# Autodesk Inventor assembly: KB33-046-002 - Привод в сборе
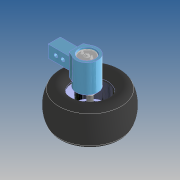
[picture p0: Inventor's stored thumbnail of the model, 180x180]
Saved by Autodesk Inventor 2020 (Build 240168000, 168)
## iProperties
Created: 2021-06-21
Part Number: KB33-046-002 - Привод в сборе
Document SubType Name: Assembly
Designer: Петров Иван
Mass: 1171.6 g
Surface Area: 1587.77 cm^2
Volume: 1165.85 cm^3
Density: 1.00493 g/cm^3
Author: Петров Иван
## Documents named in this file (6)
- E:\IVAN\Ivan_desktop\Kvantorium\Projects\RoboPatrol\design\KB33-046-002 - Привод в сборе.iam
- E:\IVAN\Ivan_desktop\Kvantorium\Projects\RoboPatrol\design\KB33-046-002-001 - Крепление.ipt
- E:\IVAN\Ivan_desktop\Kvantorium\Projects\RoboPatrol\design\standart_components\dc_gear_motor_12V_500rpm\dc_gear_motor_12V_500rpm.ipt
- E:\IVAN\Ivan_desktop\Kvantorium\Projects\RoboPatrol\design\standart_components\WheelBig\колесо большое1.iam
- E:\IVAN\Ivan_desktop\Kvantorium\Projects\RoboPatrol\design\KB33-046-002-002 - Втулка.ipt
- E:\IVAN\Ivan_desktop\Kvantorium\Projects\RoboPatrol\design\KB33-046-002-003 - Фиксирующая гайка.ipt
## Components (6 placed, 5 different names)
1. KB33-046-002-001 - Крепление:1 — Заподлицо:1, Совмещение:1, Совмещение:2
2. dc_gear_motor_12V_500rpm:1 — Заподлицо:1, Совмещение:1, Совмещение:2, Совмещение:3, Совмещение:4, Совмещение:5, Совмещение:6, Угол:1
3. колесо большое1:1 [sub-assembly] — Совмещение:3, Совмещение:4, Угол:2, Совмещение:8, Совмещение:10
4. KB33-046-002-002 - Втулка:1 — Совмещение:5, Совмещение:6, Угол:1, Совмещение:7, Совмещение:9
5. KB33-046-002-003 - Фиксирующая гайка:1 — Совмещение:7, Угол:2, Совмещение:8
6. KB33-046-002-003 - Фиксирующая гайка:2 — Совмещение:9, Совмещение:10
## Relationships (13: Mate 10, Angle 2, Flush 1)
- Заподлицо:1 [Flush]: KB33-046-002-001 - Крепление:1 ↔ dc_gear_motor_12V_500rpm:1
- Совмещение:1 [Mate]: KB33-046-002-001 - Крепление:1 ↔ dc_gear_motor_12V_500rpm:1
- Совмещение:2 [Mate]: KB33-046-002-001 - Крепление:1 ↔ dc_gear_motor_12V_500rpm:1
- Совмещение:3 [Mate] (30 mm): dc_gear_motor_12V_500rpm:1 ↔ колесо большое1:1
- Совмещение:4 [Mate]: dc_gear_motor_12V_500rpm:1 ↔ колесо большое1:1
- Совмещение:5 [Mate]: dc_gear_motor_12V_500rpm:1 ↔ KB33-046-002-002 - Втулка:1
- Совмещение:6 [Mate]: dc_gear_motor_12V_500rpm:1 ↔ KB33-046-002-002 - Втулка:1
- Угол:1 [Angle] (180 deg): dc_gear_motor_12V_500rpm:1 ↔ KB33-046-002-002 - Втулка:1
- Совмещение:7 [Mate]: KB33-046-002-002 - Втулка:1 ↔ KB33-046-002-003 - Фиксирующая гайка:1
- Угол:2 [Angle] (0 deg): колесо большое1:1 ↔ KB33-046-002-003 - Фиксирующая гайка:1
- Совмещение:8 [Mate]: колесо большое1:1 ↔ KB33-046-002-003 - Фиксирующая гайка:1
- Совмещение:9 [Mate]: KB33-046-002-002 - Втулка:1 ↔ KB33-046-002-003 - Фиксирующая гайка:2
- Совмещение:10 [Mate]: колесо большое1:1 ↔ KB33-046-002-003 - Фиксирующая гайка:2
